# Autodesk Inventor assembly: Body Assembly
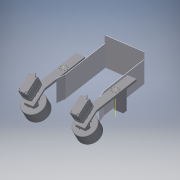
[picture p0: Inventor's stored thumbnail of the model, 180x180]
Saved by Autodesk Inventor 2019 (Build 230136000, 136)
## iProperties
Created: 2019-10-15
Part Number: Body Assembly
Document SubType Name: Assembly
Designer: User
Author: User
## Documents named in this file (14)
- C:\Robotics\CAD\2019-20_CAD\Collection\Body Assembly.iam
- C:\Robotics\CAD\2019-20_CAD\Collection\U-Part Gen 2.ipt
- C:\Robotics\CAD\2019-20_CAD\Collection\wheel arm stand off.ipt
- C:\Robotics\CAD\2019-20_CAD\Collection\arm assembaly.iam
- C:\Robotics\CAD\COTSParts\Vex\2-Wire_Motor_393_276-2177.iam
- C:\Robotics\CAD\COTSParts\Wheels\2.5inFoamWheel250TMD.ipt
- C:\Robotics\CAD\2019-20_CAD\Collection\vex motor adaptor to tetrix.ipt
- C:\Robotics\CAD\COTSParts\Bearings - AndyMark\Bearing 250 ID 500 OD flanged.ipt
- C:\Robotics\CAD\2019-20_CAD\Collection\wheel arm stand off_MIR.ipt
- C:\Robotics\CAD\2019-20_CAD\Collection\arm assembaly_MIR.iam
- C:\Robotics\CAD\COTSParts\Vex\2-Wire_Motor_393_276-2177_MIR.iam
- C:\Robotics\CAD\2019-20_CAD\Collection\vex motor adaptor to tetrix_MIR.ipt
- C:\Robotics\CAD\COTSParts\Wheels\2.5inFoamWheel250TMD_MIR.ipt
- C:\Robotics\CAD\COTSParts\Bearings - AndyMark\Bearing 250 ID 500 OD flanged_MIR1.ipt
## Components (13 placed, 13 different names)
1. U-Part Gen 2:1 — Mate:23, Flush:10, Flush:25, Flush:27, Mate:57
2. wheel arm stand off:2 — Mate:22, Mate:23, Flush:10, Flush:25, Flush:28, Flush:31, Mate:61
3. arm assembaly:1 [sub-assembly] — Mate:22, Mate:24, Mate:25, Mate:26, Mate:28, Mate:32, Flush:31, Mate:61
4. 2-Wire_Motor_393_276-2177:1 [sub-assembly] — Mate:24, Mate:25, Mate:26, Mate:27
5. vex motor adaptor to tetrix:1 — Mate:27, Mate:28, Mate:29, Insert:1, Mate:30, Mate:31
6. 2.5inFoamWheel250TMD:1 — Mate:29, Insert:1, Mate:30
7. Bearing 250 ID 500 OD flanged:1 — Mate:31, Mate:32
8. wheel arm stand off_MIR:1 — Mate:43, Flush:27, Mate:57, Flush:28, Flush:30, Mate:60
9. arm assembaly_MIR:1 [sub-assembly] — Mate:43, Mate:45, Mate:46, Mate:47, Mate:48, Mate:52, Flush:30, Mate:60
10. 2-Wire_Motor_393_276-2177_MIR:1 [sub-assembly] — Mate:45, Mate:46, Mate:47, Mate:49
11. vex motor adaptor to tetrix_MIR:1 — Mate:48, Mate:49, Mate:50, Insert:2, Mate:51, Mate:53
12. 2.5inFoamWheel250TMD_MIR:1 — Mate:50, Insert:2, Mate:51
13. Bearing 250 ID 500 OD flanged_MIR1:1 — Mate:52, Mate:53
## Relationships (32: Mate 24, Flush 6, Insert 2)
- Mate:22: wheel arm stand off:2 ↔ arm assembaly:1
- Mate:23 (4.7625 mm): U-Part Gen 2:1 ↔ wheel arm stand off:2
- Flush:10 (-108.4072 mm): U-Part Gen 2:1 ↔ wheel arm stand off:2
- Mate:24: arm assembaly:1 ↔ 2-Wire_Motor_393_276-2177:1
- Mate:25: arm assembaly:1 ↔ 2-Wire_Motor_393_276-2177:1
- Mate:26: arm assembaly:1 ↔ 2-Wire_Motor_393_276-2177:1
- Mate:27: 2-Wire_Motor_393_276-2177:1 ↔ vex motor adaptor to tetrix:1
- Mate:28: arm assembaly:1 ↔ vex motor adaptor to tetrix:1
- Mate:29: vex motor adaptor to tetrix:1 ↔ 2.5inFoamWheel250TMD:1
- Insert:1: vex motor adaptor to tetrix:1 ↔ 2.5inFoamWheel250TMD:1
- Mate:30: vex motor adaptor to tetrix:1 ↔ 2.5inFoamWheel250TMD:1
- Mate:31: vex motor adaptor to tetrix:1 ↔ Bearing 250 ID 500 OD flanged:1
- Mate:32: arm assembaly:1 ↔ Bearing 250 ID 500 OD flanged:1
- Mate:43: wheel arm stand off_MIR:1 ↔ arm assembaly_MIR:1
- Mate:45: arm assembaly_MIR:1 ↔ 2-Wire_Motor_393_276-2177_MIR:1
- Mate:46: arm assembaly_MIR:1 ↔ 2-Wire_Motor_393_276-2177_MIR:1
- Mate:47: arm assembaly_MIR:1 ↔ 2-Wire_Motor_393_276-2177_MIR:1
- Mate:48: arm assembaly_MIR:1 ↔ vex motor adaptor to tetrix_MIR:1
- Mate:49: 2-Wire_Motor_393_276-2177_MIR:1 ↔ vex motor adaptor to tetrix_MIR:1
- Mate:50: vex motor adaptor to tetrix_MIR:1 ↔ 2.5inFoamWheel250TMD_MIR:1
- Insert:2: vex motor adaptor to tetrix_MIR:1 ↔ 2.5inFoamWheel250TMD_MIR:1
- Mate:51: vex motor adaptor to tetrix_MIR:1 ↔ 2.5inFoamWheel250TMD_MIR:1
- Mate:52: arm assembaly_MIR:1 ↔ Bearing 250 ID 500 OD flanged_MIR1:1
- Mate:53: vex motor adaptor to tetrix_MIR:1 ↔ Bearing 250 ID 500 OD flanged_MIR1:1
- Flush:25: U-Part Gen 2:1 ↔ wheel arm stand off:2
- Flush:27: U-Part Gen 2:1 ↔ wheel arm stand off_MIR:1
- Mate:57 (4.7625 mm): U-Part Gen 2:1 ↔ wheel arm stand off_MIR:1
- Flush:28: wheel arm stand off:2 ↔ wheel arm stand off_MIR:1
- Flush:30: wheel arm stand off_MIR:1 ↔ arm assembaly_MIR:1
- Mate:60: wheel arm stand off_MIR:1 ↔ arm assembaly_MIR:1
- Flush:31: wheel arm stand off:2 ↔ arm assembaly:1
- Mate:61: wheel arm stand off:2 ↔ arm assembaly:1
